# Autodesk Inventor assembly: ASSEMBLY_Main
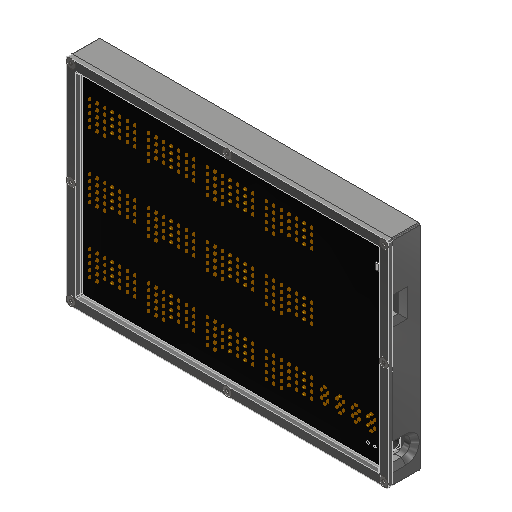
[picture p0: Inventor's stored thumbnail of the model, 512x512]
Saved by Autodesk Inventor 2025 (Build 290162010, 162A)
## iProperties
Created: 2024-08-15
Part Number: ASSEMBLY_Main
Document SubType Name: Assembly
Designer: User
Author: User
## Documents named in this file (11)
- D:\_ANDRZEJ_LACZEWSKI\_OTHER\ELECTR - LED Calendar\MCAD\ASSEMBLY_MAIN_REVA\ASSEMBLY_Main.iam
- D:\_ANDRZEJ_LACZEWSKI\_OTHER\ELECTR - LED Calendar\MCAD\ASSEMBLY_MAIN_REVA\3DP_PLA_Back_Cover.ipt
- D:\_ANDRZEJ_LACZEWSKI\_OTHER\ELECTR - LED Calendar\MCAD\__ALTIUM_PCB_PARTS\PCB_LED_CALENDAR\PCB_LED_CALENDAR.iam
- D:\_ANDRZEJ_LACZEWSKI\_OTHER\ELECTR - LED Calendar\MCAD\ASSEMBLY_MAIN_REVA\3DP_PLA_Front_Mounting_Bracket.ipt
- D:\_ANDRZEJ_LACZEWSKI\_OTHER\ELECTR - LED Calendar\MCAD\__CONTENT_CENTER_PARTS\DIN 7991(2)\DIN 7991 - M3x12.ipt
- D:\_ANDRZEJ_LACZEWSKI\_OTHER\ELECTR - LED Calendar\MCAD\ASSEMBLY_MAIN_REVA\3DP_PLA_Stand_Leg_Mount.ipt
- D:\_ANDRZEJ_LACZEWSKI\_OTHER\ELECTR - LED Calendar\MCAD\ASSEMBLY_MAIN_REVA\3DP_PLA_Stand_Leg.ipt
- D:\_ANDRZEJ_LACZEWSKI\_OTHER\ELECTR - LED Calendar\MCAD\__CONTENT_CENTER_PARTS\DIN 7991(2)\DIN 7991 - M3x8.ipt
- D:\_ANDRZEJ_LACZEWSKI\_OTHER\ELECTR - LED Calendar\MCAD\__CONTENT_CENTER_PARTS\DIN 125-2  A\DIN 125-2 - A 3,2A.ipt
- D:\_ANDRZEJ_LACZEWSKI\_OTHER\ELECTR - LED Calendar\MCAD\__CONTENT_CENTER_PARTS\ISO 7380-1\ISO 7380-1 - M3 x 30.ipt
- D:\_ANDRZEJ_LACZEWSKI\_OTHER\ELECTR - LED Calendar\MCAD\__CONTENT_CENTER_PARTS\DIN 934\DIN 934 - M3 x 0,5.ipt
## Components (31 placed, 10 different names)
1. 3DP_PLA_Back_Cover:1 — Mate:1, Mate:2, Mate:3, Mate:4, Flush:1, Flush:2, Mate:13, Mate:16, Mate:17, Angle:1
2. PCB_LED_CALENDAR:1 [sub-assembly] — Mate:1, Mate:2, Mate:3
3. 3DP_PLA_Front_Mounting_Bracket:1 — Mate:4, Flush:1, Flush:2, Mate:5, Mate:6, Mate:7, Mate:8, Mate:9, Mate:10, Mate:11, Mate:12
4. 3DP_PLA_Stand_Leg_Mount:1 — Mate:13, Mate:14, Mate:15, Mate:16, Mate:17, Mate:18, Mate:19, Mate:20, Mate:21, Mate:22, Mate:23, Mate:24, Mate:25, Mate:26, Mate:27, Mate:28, Mate:29, Mate:30, Mate:31
5. 3DP_PLA_Stand_Leg:1 — Mate:14, Mate:15, Mate:34, Mate:35, Mate:38, Mate:39, Angle:1
6. DIN 125-2 A A 3,2:8 — Mate:37, Mate:38
7. DIN 125-2 A A 3,2:7 — Mate:36, Mate:39
8. DIN 125-2 A A 3,2:6 — Mate:33, Mate:34
9. DIN 125-2 A A 3,2:5 — Mate:32, Mate:35
10. DIN 934 - replaced by DIN EN 24032/28673/28674 M3:2 — Insert:4
11. DIN 125-2 A A 3,2:4 — Mate:30, Mate:31, Insert:4
12. ISO 7380-1 M3 x 30:2 — Insert:3, Mate:36, Mate:37
13. DIN 125-2 A A 3,2:3 — Mate:28, Mate:29, Insert:3
14. DIN 934 - replaced by DIN EN 24032/28673/28674 M3:1 — Insert:2
15. DIN 125-2 A A 3,2:2 — Mate:26, Mate:27, Insert:2
16. ISO 7380-1 M3 x 30:1 — Insert:1, Mate:32, Mate:33
17. DIN 125-2 A A 3,2:1 — Mate:24, Mate:25, Insert:1
18. DIN 7991 M3x12:1 — Mate:5
19. DIN 7991 M3x8:1 — Mate:18
20. DIN 7991 M3x8:2 — Mate:19
21. DIN 7991 M3x8:3 — Mate:20
22. DIN 7991 M3x8:4 — Mate:21
23. DIN 7991 M3x8:5 — Mate:22
24. DIN 7991 M3x8:6 — Mate:23
25. DIN 7991 M3x12:2 — Mate:6
26. DIN 7991 M3x12:3 — Mate:7
27. DIN 7991 M3x12:4 — Mate:8
28. DIN 7991 M3x12:5 — Mate:9
29. DIN 7991 M3x12:6 — Mate:10
30. DIN 7991 M3x12:7 — Mate:11
31. DIN 7991 M3x12:8 — Mate:12
## Relationships (46: Mate 39, Insert 4, Flush 2, Angle 1)
- Mate:1: 3DP_PLA_Back_Cover:1 ↔ PCB_LED_CALENDAR:1
- Mate:2 (0.5 mm): 3DP_PLA_Back_Cover:1 ↔ PCB_LED_CALENDAR:1
- Mate:3 (0.5 mm): 3DP_PLA_Back_Cover:1 ↔ PCB_LED_CALENDAR:1
- Mate:4: 3DP_PLA_Back_Cover:1 ↔ 3DP_PLA_Front_Mounting_Bracket:1
- Flush:1: 3DP_PLA_Back_Cover:1 ↔ 3DP_PLA_Front_Mounting_Bracket:1
- Flush:2: 3DP_PLA_Back_Cover:1 ↔ 3DP_PLA_Front_Mounting_Bracket:1
- Mate:5: 3DP_PLA_Front_Mounting_Bracket:1 ↔ DIN 7991 M3x12:1
- Mate:6: 3DP_PLA_Front_Mounting_Bracket:1 ↔ DIN 7991 M3x12:2
- Mate:7: 3DP_PLA_Front_Mounting_Bracket:1 ↔ DIN 7991 M3x12:3
- Mate:8: 3DP_PLA_Front_Mounting_Bracket:1 ↔ DIN 7991 M3x12:4
- Mate:9: 3DP_PLA_Front_Mounting_Bracket:1 ↔ DIN 7991 M3x12:5
- Mate:10: 3DP_PLA_Front_Mounting_Bracket:1 ↔ DIN 7991 M3x12:6
- Mate:11: 3DP_PLA_Front_Mounting_Bracket:1 ↔ DIN 7991 M3x12:7
- Mate:12: 3DP_PLA_Front_Mounting_Bracket:1 ↔ DIN 7991 M3x12:8
- Mate:13: 3DP_PLA_Back_Cover:1 ↔ 3DP_PLA_Stand_Leg_Mount:1
- Mate:14: 3DP_PLA_Stand_Leg_Mount:1 ↔ 3DP_PLA_Stand_Leg:1
- Mate:15 (0.5 mm): 3DP_PLA_Stand_Leg_Mount:1 ↔ 3DP_PLA_Stand_Leg:1
- Mate:16: 3DP_PLA_Back_Cover:1 ↔ 3DP_PLA_Stand_Leg_Mount:1
- Mate:17: 3DP_PLA_Back_Cover:1 ↔ 3DP_PLA_Stand_Leg_Mount:1
- Mate:18: 3DP_PLA_Stand_Leg_Mount:1 ↔ DIN 7991 M3x8:1
- Mate:19: 3DP_PLA_Stand_Leg_Mount:1 ↔ DIN 7991 M3x8:2
- Mate:20: 3DP_PLA_Stand_Leg_Mount:1 ↔ DIN 7991 M3x8:3
- Mate:21: 3DP_PLA_Stand_Leg_Mount:1 ↔ DIN 7991 M3x8:4
- Mate:22: 3DP_PLA_Stand_Leg_Mount:1 ↔ DIN 7991 M3x8:5
- Mate:23: 3DP_PLA_Stand_Leg_Mount:1 ↔ DIN 7991 M3x8:6
- Mate:24: 3DP_PLA_Stand_Leg_Mount:1 ↔ DIN 125-2 A A 3,2:1
- Mate:25: 3DP_PLA_Stand_Leg_Mount:1 ↔ DIN 125-2 A A 3,2:1
- Insert:1: ISO 7380-1 M3 x 30:1 ↔ DIN 125-2 A A 3,2:1
- Mate:26: 3DP_PLA_Stand_Leg_Mount:1 ↔ DIN 125-2 A A 3,2:2
- Mate:27: 3DP_PLA_Stand_Leg_Mount:1 ↔ DIN 125-2 A A 3,2:2
- Insert:2: DIN 934 - replaced by DIN EN 24032/28673/28674 M3:1 ↔ DIN 125-2 A A 3,2:2
- Mate:28: 3DP_PLA_Stand_Leg_Mount:1 ↔ DIN 125-2 A A 3,2:3
- Mate:29: 3DP_PLA_Stand_Leg_Mount:1 ↔ DIN 125-2 A A 3,2:3
- Insert:3: ISO 7380-1 M3 x 30:2 ↔ DIN 125-2 A A 3,2:3
- Mate:30: 3DP_PLA_Stand_Leg_Mount:1 ↔ DIN 125-2 A A 3,2:4
- Mate:31: 3DP_PLA_Stand_Leg_Mount:1 ↔ DIN 125-2 A A 3,2:4
- Insert:4: DIN 934 - replaced by DIN EN 24032/28673/28674 M3:2 ↔ DIN 125-2 A A 3,2:4
- Mate:32: DIN 125-2 A A 3,2:5 ↔ ISO 7380-1 M3 x 30:1
- Mate:33: DIN 125-2 A A 3,2:6 ↔ ISO 7380-1 M3 x 30:1
- Mate:34: 3DP_PLA_Stand_Leg:1 ↔ DIN 125-2 A A 3,2:6
- Mate:35: 3DP_PLA_Stand_Leg:1 ↔ DIN 125-2 A A 3,2:5
- Mate:36: DIN 125-2 A A 3,2:7 ↔ ISO 7380-1 M3 x 30:2
- Mate:37: DIN 125-2 A A 3,2:8 ↔ ISO 7380-1 M3 x 30:2
- Mate:38: 3DP_PLA_Stand_Leg:1 ↔ DIN 125-2 A A 3,2:8
- Mate:39: 3DP_PLA_Stand_Leg:1 ↔ DIN 125-2 A A 3,2:7
- Angle:1 (0 deg): 3DP_PLA_Back_Cover:1 ↔ 3DP_PLA_Stand_Leg:1
